# Autodesk Inventor assembly: TR2 Arm
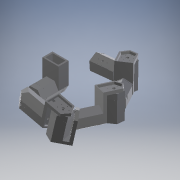
[picture p0: Inventor's stored thumbnail of the model, 180x180]
Saved by Autodesk Inventor 2017 (Build 210142000, 142)
## iProperties
Created: 2018-10-11
Part Number: TR2 Arm
Document SubType Name: Assembly
Designer: Zach
Author: Zach
## Documents named in this file (5)
- C:\Users\Dell\Documents\GitHub\tr2\Arm\Arm.iam
- C:\Users\Dell\Documents\GitHub\tr2\Arm\TARM01.ipt
- C:\Users\Dell\Documents\GitHub\tr2\Arm Actuator\Arm Actuator.iam
- C:\Users\Dell\Documents\GitHub\tr2\Arm\TARM02.ipt
- C:\Users\Dell\Documents\GitHub\tr2\Arm\TARM03.ipt
## Components (13 placed, 4 different names)
1. TARM01:1 — Mate:9, Mate:10, Mate:11
2. TARM02:1 — Mate:13, Mate:19, Mate:20, Mate:43, Mate:44
3. TARM03:1 — Mate:20, Mate:23, Mate:24, Mate:43, Mate:44
4. TARM03:2 — Mate:33, Mate:34, Mate:35
5. Arm Actuator:1 [sub-assembly] — Mate:9, Mate:10, Mate:11, Mate:13, Mate:19
6. Arm Actuator:2 [sub-assembly] — Mate:23, Mate:24, Mate:27, Mate:28, Mate:45, Mate:46, Mate:47
7. Arm Actuator:3 [sub-assembly] — Mate:27, Mate:28, Mate:33, Mate:34, Mate:35
8. Arm Actuator:4 [sub-assembly]
9. Arm Actuator:5 [sub-assembly] — Mate:40, Mate:41, Mate:42
10. TARM03:3 — Mate:40, Mate:41, Mate:42
11. Arm Actuator:6 [sub-assembly]
12. Arm Actuator:7 [sub-assembly]
13. TARM03:4 — Mate:45, Mate:46, Mate:47
## Relationships (29: Mate 29)
- Mate:9: TARM01:1 ↔ Arm Actuator:1
- Mate:10: TARM01:1 ↔ Arm Actuator:1
- Mate:11: TARM01:1 ↔ Arm Actuator:1
- Mate:13: TARM02:1 ↔ Arm Actuator:1
- Mate:19: TARM02:1 ↔ Arm Actuator:1
- Mate:20: TARM02:1 ↔ TARM03:1
- Mate:23: TARM03:1 ↔ Arm Actuator:2
- Mate:24: TARM03:1 ↔ Arm Actuator:2
- Mate:27: Arm Actuator:2 ↔ Arm Actuator:3
- Mate:28: Arm Actuator:2 ↔ Arm Actuator:3
- [Mate]: TARM03:2 ↔ Arm Actuator:4
- [Mate]: TARM03:2 ↔ Arm Actuator:4
- [Mate]: Arm Actuator:4 ↔ Arm Actuator:5
- [Mate]: Arm Actuator:4 ↔ Arm Actuator:5
- Mate:33: TARM03:2 ↔ Arm Actuator:3
- Mate:34: TARM03:2 ↔ Arm Actuator:3
- Mate:35: TARM03:2 ↔ Arm Actuator:3
- [Mate]: TARM03:3 ↔ Arm Actuator:6
- [Mate]: TARM03:3 ↔ Arm Actuator:6
- [Mate]: Arm Actuator:6 ↔ Arm Actuator:7
- [Mate]: Arm Actuator:6 ↔ Arm Actuator:7
- Mate:40: Arm Actuator:5 ↔ TARM03:3
- Mate:41: Arm Actuator:5 ↔ TARM03:3
- Mate:42: Arm Actuator:5 ↔ TARM03:3
- Mate:43: TARM02:1 ↔ TARM03:1
- Mate:44: TARM02:1 ↔ TARM03:1
- Mate:45: Arm Actuator:2 ↔ TARM03:4
- Mate:46: Arm Actuator:2 ↔ TARM03:4
- Mate:47: Arm Actuator:2 ↔ TARM03:4
## Named parameters: d84_d82 = 0 mm, d85_d83 = 0 mm, d86_d78 = 0 mm, d87_d79 = 0 mm, d91_d84_d82 = 0 mm, d92_d85_d83 = 0 mm, d93_d86_d78 = 0 mm, d94_d87_d79 = 0 mm
